# Autodesk Inventor assembly: Assembly_SIMMO_1
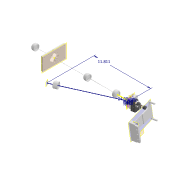
[picture p0: Inventor's stored thumbnail of the model, 180x180]
Saved by Autodesk Inventor 2022 (Build 260153000, 153)
## iProperties
Created: 2022-04-09
Part Number: Assembly_SIMMO_1
Document SubType Name: Assembly
Designer: Prakash Lab
Author: Prakash Lab
## Documents named in this file (10)
- E:\GitHub\SIMMO\INVENTOR\Assembly_SIMMO_1.iam
- E:\GitHub\SIMMO\INVENTOR\00_AC254-200-A-ML-Step.ipt
- E:\GitHub\SIMMO\INVENTOR\Adapter_DMD_KM100.ipt
- E:\GitHub\SIMMO\INVENTOR\Cover_new.ipt
- E:\GitHub\SIMMO\INVENTOR\KM100-Solidworks.ipt
- E:\GitHub\SIMMO\INVENTOR\Mount_new.ipt
- E:\GitHub\SIMMO\INVENTOR\Nikon_Ti2E.ipt
- E:\GitHub\SIMMO\INVENTOR\00_AC254-030-A-ML-Step.ipt
- E:\GitHub\SIMMO\INVENTOR\00_AC254-075-A-ML-Step.ipt
- E:\GitHub\SIMMO\INVENTOR\00_Beampath_v0.ipt
## Components (10 placed, 9 different names)
1. Adapter_DMD_KM100:1 — Insert:5, Mate:5, Insert:6, Mate:6
2. KM100-Solidworks:1 — Insert:6, Angle:3
3. Mount_new:1 — Mate:6
4. 00_AC254-030-A-ML-Step:1 — Insert:4
5. Nikon_Ti2E:1 — Mate:1, Mate:2, Mate:3, Flush:1, Flush:2
6. 00_Beampath_v0:1 — Flush:1, Flush:2, Insert:1, Insert:2, Insert:3, Angle:1, Mate:4, Insert:4
7. 00_AC254-200-A-ML-Step:1 — Insert:1
8. 00_AC254-075-A-ML-Step:1 — Insert:2
9. 00_AC254-075-A-ML-Step:2 — Insert:3
10. Cover_new:1 — Angle:1, Mate:4, Angle:2, Insert:5, Mate:5
## Relationships (17: Mate 6, Insert 6, Angle 3, Flush 2)
- Mate:1: Nikon_Ti2E:1
- Mate:2: Nikon_Ti2E:1
- Mate:3: Nikon_Ti2E:1
- Flush:1: Nikon_Ti2E:1 ↔ 00_Beampath_v0:1
- Flush:2: Nikon_Ti2E:1 ↔ 00_Beampath_v0:1
- Insert:1: 00_Beampath_v0:1 ↔ 00_AC254-200-A-ML-Step:1
- Insert:2: 00_Beampath_v0:1 ↔ 00_AC254-075-A-ML-Step:1
- Insert:3: 00_Beampath_v0:1 ↔ 00_AC254-075-A-ML-Step:2
- Angle:1 (190 deg): 00_Beampath_v0:1 ↔ Cover_new:1
- Mate:4: 00_Beampath_v0:1 ↔ Cover_new:1
- Angle:2 (0 deg): Cover_new:1
- Insert:4 (-30 mm): 00_AC254-030-A-ML-Step:1 ↔ 00_Beampath_v0:1
- Insert:5 (5 mm): Adapter_DMD_KM100:1 ↔ Cover_new:1
- Mate:5: Adapter_DMD_KM100:1 ↔ Cover_new:1
- Insert:6 (8 mm): Adapter_DMD_KM100:1 ↔ KM100-Solidworks:1
- Mate:6 (20 mm): Adapter_DMD_KM100:1 ↔ Mount_new:1
- Angle:3 (0 deg): KM100-Solidworks:1
